# Autodesk Inventor assembly: BBM Staging Plate Assembly
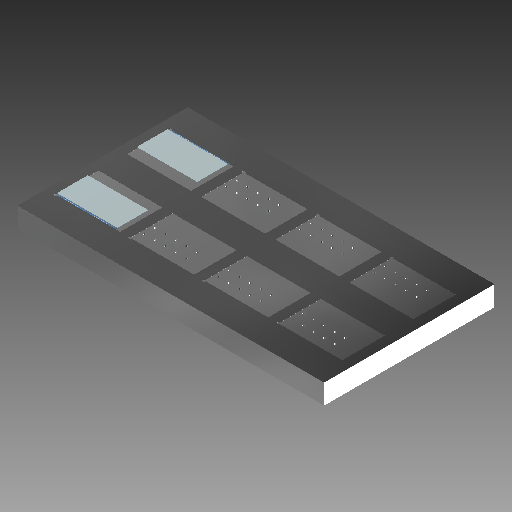
[picture p0: Inventor's stored thumbnail of the model, 512x512]
Saved by Autodesk Inventor 2019.4 (Build 234330000, 330)
## iProperties
Created: 2021-01-11
Part Number: BBM Staging Plate Assembly
Document SubType Name: Assembly
Designer: caleb
Author: caleb
## Documents named in this file (4)
- C:\Users\cfang\Desktop\nebraska-silicon-lab\Hardware\ETL\Module Assembly\BBM Staging Plate\BBM Staging Plate Assembly.iam
- C:\Users\cfang\Desktop\nebraska-silicon-lab\Hardware\ETL\Module Assembly\BBM Staging Plate\BBM Staging Plate.ipt
- C:\Users\cfang\Desktop\nebraska-silicon-lab\Hardware\ETL\Module Assembly\BBM Staging Plate\BBM Staging Plate Stencil.ipt
- C:\Users\cfang\Desktop\nebraska-silicon-lab\Hardware\ETL\Module Assembly\BBM Staging Plate\Bare Bump-Bonded Module.iam
## Components (4 placed, 3 different names)
1. BBM Staging Plate:1 — Mate:1, Flush:1, Flush:2, Mate:2, Mate:5
2. BBM Staging Plate Stencil:1 — Mate:1, Flush:1, Flush:2, Mate:3, Mate:4, Mate:6, Mate:7
3. Bare Bump-Bonded Module:4 [sub-assembly] — Mate:2, Mate:3, Mate:4
4. Bare Bump-Bonded Module:5 [sub-assembly] — Mate:5, Mate:6, Mate:7
## Relationships (9: Mate 7, Flush 2)
- Mate:1: BBM Staging Plate:1 ↔ BBM Staging Plate Stencil:1
- Flush:1: BBM Staging Plate:1 ↔ BBM Staging Plate Stencil:1
- Flush:2: BBM Staging Plate:1 ↔ BBM Staging Plate Stencil:1
- Mate:2: BBM Staging Plate:1 ↔ Bare Bump-Bonded Module:4
- Mate:3: BBM Staging Plate Stencil:1 ↔ Bare Bump-Bonded Module:4
- Mate:4: BBM Staging Plate Stencil:1 ↔ Bare Bump-Bonded Module:4
- Mate:5: BBM Staging Plate:1 ↔ Bare Bump-Bonded Module:5
- Mate:6: BBM Staging Plate Stencil:1 ↔ Bare Bump-Bonded Module:5
- Mate:7: BBM Staging Plate Stencil:1 ↔ Bare Bump-Bonded Module:5
